# Autodesk Inventor assembly: CIRCULO_OBSTRUCCION_VISUAL
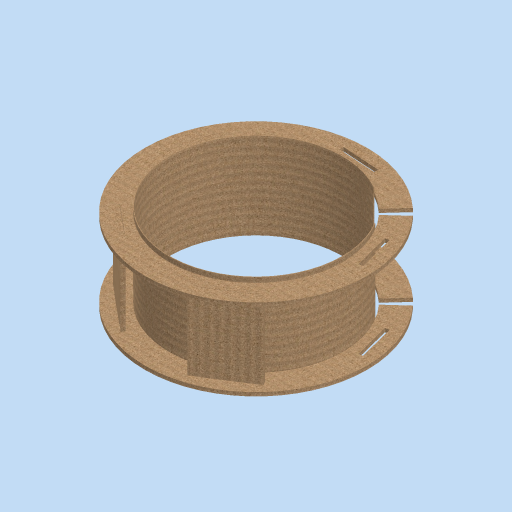
[picture p0: Inventor's stored thumbnail of the model, 512x512]
Saved by Autodesk Inventor 2024.2 (Build 282272000, 272)
## iProperties
Created: 2024-11-17
Part Number: CIRCULO_OBSTRUCCION_VISUAL
Document SubType Name: Assembly
Designer: jrcer
Author: jrcer
## Documents named in this file (4)
- C:\Users\jrcer\Universidad\S10_2024\TDG\Tesis\Modelos\CIRCULO_OBSTRUCCION_VISUAL.iam
- C:\Users\jrcer\Universidad\S10_2024\TDG\Tesis\Modelos\D14_CM_CIRCULO.ipt
- C:\Users\jrcer\Universidad\S10_2024\TDG\Tesis\Modelos\UNION_SOPORTE.ipt
- C:\Users\jrcer\Universidad\S10_2024\TDG\Tesis\Modelos\OBSTRUCCION_VISUAL.ipt
## Components (6 placed, 3 different names)
1. D14_CM_CIRCULO:1 — Mate:7, Mate:8, Flush:4, Flush:5
2. D14_CM_CIRCULO:2 — Mate:1, Flush:1, Mate:2, Mate:3, Flush:2, Mate:4, Mate:5, Flush:3, Mate:6, Mate:9
3. UNION_SOPORTE:1 — Mate:3, Flush:2, Mate:4, Mate:7, Mate:8, Flush:4
4. UNION_SOPORTE:2 — Mate:1, Flush:1, Mate:2
5. UNION_SOPORTE:3 — Mate:5, Flush:3, Mate:6
6. OBSTRUCCION_VISUAL:1 — Mate:9, Flush:5
## Relationships (14: Mate 9, Flush 5)
- Mate:1: D14_CM_CIRCULO:2 ↔ UNION_SOPORTE:2
- Flush:1: D14_CM_CIRCULO:2 ↔ UNION_SOPORTE:2
- Mate:2: D14_CM_CIRCULO:2 ↔ UNION_SOPORTE:2
- Mate:3: D14_CM_CIRCULO:2 ↔ UNION_SOPORTE:1
- Flush:2: D14_CM_CIRCULO:2 ↔ UNION_SOPORTE:1
- Mate:4: D14_CM_CIRCULO:2 ↔ UNION_SOPORTE:1
- Mate:5: D14_CM_CIRCULO:2 ↔ UNION_SOPORTE:3
- Flush:3: D14_CM_CIRCULO:2 ↔ UNION_SOPORTE:3
- Mate:6: D14_CM_CIRCULO:2 ↔ UNION_SOPORTE:3
- Mate:7: D14_CM_CIRCULO:1 ↔ UNION_SOPORTE:1
- Mate:8: D14_CM_CIRCULO:1 ↔ UNION_SOPORTE:1
- Flush:4: D14_CM_CIRCULO:1 ↔ UNION_SOPORTE:1
- Mate:9: D14_CM_CIRCULO:2 ↔ OBSTRUCCION_VISUAL:1
- Flush:5: D14_CM_CIRCULO:1 ↔ OBSTRUCCION_VISUAL:1
